# Autodesk Inventor assembly: MG-Encoderplatine
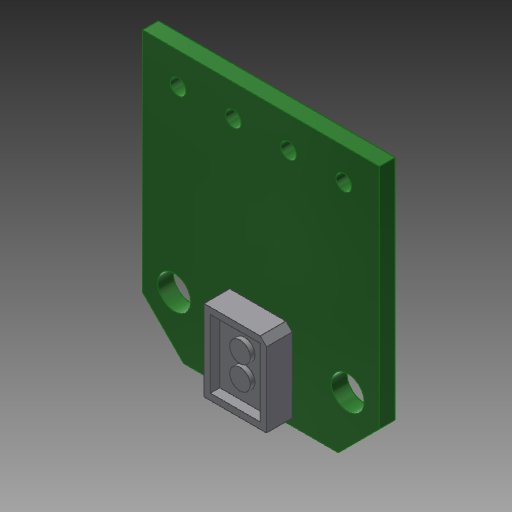
[picture p0: Inventor's stored thumbnail of the model, 512x512]
Saved by Autodesk Inventor 2019.4 (Build 234330000, 330)
## iProperties
Part Number: MG-Encoderplatine
Material: Generisch
Document SubType Name: Assembly
Designer: rYan
Mass: 0.362061 g
Surface Area: 6.73753 cm^2
Volume: 0.271556 cm^3
Density: 1.33328 g/cm^3
Author: rYan
## Documents named in this file (4)
- D:\TIGERsGIT\Hardware\mechanik\2020\Inventor\Robot\Drive Train\MG-Encoderplatine.iam
- D:\TIGERsGIT\Hardware\mechanik\2020\Inventor\Robot\Drive Train\Encoderplatine.ipt
- D:\TIGERsGIT\Hardware\mechanik\2020\Inventor\Purchased Parts\AEDR-8300-1Wx Encoder.ipt
- D:\TIGERsGIT\Hardware\mechanik\2020\Inventor\Purchased Parts\iC-PX Series Encoder.ipt
## Components (3 placed, 3 different names)
1. Encoderplatine:1 — Passend:1, Fluchtend:1, Fluchtend:2, Passend:2, Fluchtend:3, Fluchtend:4
2. AEDR-8300-1Wx Encoder:1 — Passend:1, Fluchtend:1, Fluchtend:2
3. iC-PX Series Encoder:1 — Passend:2, Fluchtend:3, Fluchtend:4
## Relationships (6: Flush 4, Mate 2)
- Passend:1 [Mate]: Encoderplatine:1 ↔ AEDR-8300-1Wx Encoder:1
- Fluchtend:1 [Flush] (0.44 mm): Encoderplatine:1 ↔ AEDR-8300-1Wx Encoder:1
- Fluchtend:2 [Flush]: Encoderplatine:1 ↔ AEDR-8300-1Wx Encoder:1
- Passend:2 [Mate]: Encoderplatine:1 ↔ iC-PX Series Encoder:1
- Fluchtend:3 [Flush]: Encoderplatine:1 ↔ iC-PX Series Encoder:1
- Fluchtend:4 [Flush] (-1.581 mm): Encoderplatine:1 ↔ iC-PX Series Encoder:1
